# Autodesk Inventor assembly: Сборка1
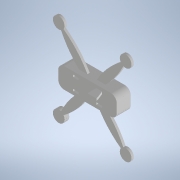
[picture p0: Inventor's stored thumbnail of the model, 180x180]
Saved by Autodesk Inventor 2022 (Build 260153000, 153)
## iProperties
Created: 2025-06-24
Part Number: Сборка1
Document SubType Name: Assembly
Designer: korsh524
Author: korsh524
## Documents named in this file (9)
- C:\git\Olymp20205Smena\Dezign\Drone\Сборка1.iam
- C:\git\Olymp20205Smena\Dezign\Drone\Dron.ipt
- C:\git\Olymp20205Smena\Dezign\Drone\bth.ipt
- C:\git\Olymp20205Smena\Dezign\Drone\top.ipt
- C:\git\Olymp20205Smena\Dezign\Drone\top2.ipt
- C:\git\Olymp20205Smena\Dezign\Drone\topzagl.ipt
- C:\git\Olymp20205Smena\Dezign\Drone\foot.ipt
- C:\git\Olymp20205Smena\Dezign\Drone\footbtn.ipt
- C:\git\Olymp20205Smena\Dezign\Drone\ring.ipt
## Components (10 placed, 8 different names)
1. Dron:1 — Заподлицо:1, Совмещение:2, Заподлицо:4, Заподлицо:5, Заподлицо:12
2. bth:1 — Заподлицо:1, Совмещение:1, Заподлицо:2, Заподлицо:3
3. bth:2 — Совмещение:1, Заподлицо:2, Заподлицо:3, Заподлицо:11
4. top:1 — Совмещение:2, Заподлицо:4, Заподлицо:5, Совмещение:3, Заподлицо:7
5. top:2 — Совмещение:3, Заподлицо:7, Заподлицо:8
6. top2:1 — Заподлицо:8, Заподлицо:9, Заподлицо:10
7. topzagl:1 — Заподлицо:9, Заподлицо:10
8. foot:1
9. footbtn:1 — Заподлицо:11
10. ring:1 — Заподлицо:12
## Relationships (14: Flush 11, Mate 3)
- Заподлицо:1 [Flush]: Dron:1 ↔ bth:1
- Совмещение:1 [Mate]: bth:1 ↔ bth:2
- Заподлицо:2 [Flush]: bth:1 ↔ bth:2
- Заподлицо:3 [Flush]: bth:1 ↔ bth:2
- Совмещение:2 [Mate]: Dron:1 ↔ top:1
- Заподлицо:4 [Flush]: Dron:1 ↔ top:1
- Заподлицо:5 [Flush]: Dron:1 ↔ top:1
- Совмещение:3 [Mate]: top:1 ↔ top:2
- Заподлицо:7 [Flush]: top:1 ↔ top:2
- Заподлицо:8 [Flush]: top:2 ↔ top2:1
- Заподлицо:9 [Flush]: top2:1 ↔ topzagl:1
- Заподлицо:10 [Flush]: top2:1 ↔ topzagl:1
- Заподлицо:11 [Flush]: bth:2 ↔ footbtn:1
- Заподлицо:12 [Flush]: Dron:1 ↔ ring:1
